# Autodesk Inventor assembly: D20
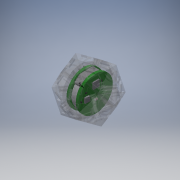
[picture p0: Inventor's stored thumbnail of the model, 180x180]
Saved by Autodesk Inventor 2019.4 (Build 234330000, 330)
## iProperties
Created: 2020-05-11
Part Number: D20
Document SubType Name: Assembly
Designer: Jorian Brusind
Author: Jorian Brusind
## Documents named in this file (5)
- C:\Users\Jorian Brusind\Documents\GitHub\PersonalProjects\DND\Dice\D20.iam
- C:\Users\Jorian Brusind\Documents\GitHub\PersonalProjects\DND\Dice\D20_lower_half.ipt
- C:\Users\Jorian Brusind\Documents\GitHub\PersonalProjects\DND\Dice\D20_upper_half.ipt
- C:\Users\Jorian Brusind\Documents\GitHub\PersonalProjects\DND\Dice\Light-Up D20\ExportSTEP\Main.iam
- C:\Users\Jorian Brusind\Documents\GitHub\PersonalProjects\DND\Dice\Light-Up D20\ExportSTEP\Main_2.iam
## Components (4 placed, 4 different names)
1. D20_lower_half:1 — Mate:2, Flush:1, Flush:2, Mate:3
2. D20_upper_half:1 — Flush:1, Flush:2, Mate:3, Mate:4, Mate:5, Mate:7
3. Main:1 [sub-assembly] — Mate:4, Mate:5, Mate:6
4. Main_2:1 [sub-assembly] — Mate:6, Mate:7
## Relationships (8: Mate 6, Flush 2)
- Mate:2: D20_lower_half:1
- Flush:1: D20_lower_half:1 ↔ D20_upper_half:1
- Flush:2: D20_lower_half:1 ↔ D20_upper_half:1
- Mate:3: D20_lower_half:1 ↔ D20_upper_half:1
- Mate:4 (1 mm): D20_upper_half:1 ↔ Main:1
- Mate:5: D20_upper_half:1 ↔ Main:1
- Mate:6 (0.25 mm): Main:1 ↔ Main_2:1
- Mate:7: D20_upper_half:1 ↔ Main_2:1
